# Autodesk Inventor assembly: JKSG10-95-S1
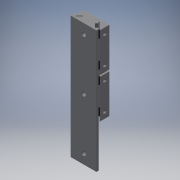
[picture p0: Inventor's stored thumbnail of the model, 180x180]
Saved by Autodesk Inventor 2019 (Build 230136000, 136)
## iProperties
Category: PARTsolutions
Company: MISUMI
Created: 2024-06-28
Part Number: JKSG10-95-S1
Catalog Web Link: www.cadenas.de
Description: JKSG, JKSC-Simplified Slide Guides for Jigs - Bearing Type Sets
Vendor: MISUMI
Document SubType Name: Assembly
Designer: psAdmin
Manufacturer: MISUMI
Mass: 13.3449 g
Surface Area: 105.666 cm^2
Volume: 13.3449 cm^3
Density: 1 g/cm^3
Title: JKSG10-95-S1
Author: Cadenas PARTsolutions
Comments: Simplified Slide Guides for Jigs - Bearing Type Sets
PSOL_IDENT_0: {$CADENAS_DATA/23d-libs/misumi/metric/07_slide_rails/jksg_asmtab.prj},205 {VTYP=3D},{STYP=ASSTAB},{N
PSOL_IDENT_1: B=JKSG10-95-S1},{LINA=JKSG10-95-S1},{NN=JKSG, JKSC},{DATE=30.06.2023 07:10:19},{GEOMDATE=09.06.2023
PSOL_IDENT_2: 02:21:08},{VERSION=},{LINEID=10},{WBVAR=TS,L,ALT,S,CALT},{WBNUMERIC=L,S,CALT}  {NB=JKSG10-95-S1},{LI
PSOL_IDENT_3: NA=JKSG10-95-S1},{KT=DUMMY},{PN=JKSG10-95-S1},{TS=SG},{L=95},{MATR=Aluminum},{MATB=Aluminum},{MATT=3
PSOL_IDENT_4: 03 Stainless Steel},{MATTP=Polyacetal},{STB=Hard Alumite Treatment},{STR=Hard Alumite Treatment},{H=
PSOL_IDENT_5: 10},{HALG=10},{A=20},{B=30},{P1=13},{P2=13},{M=3},{MALG= 'M3','M3' },{M1=3},{C=24.0},{D=6},{H1=7.5},
PSOL_IDENT_6: {E=1.8},{DGH=3.5X6X4},{N=7.5},{P=40},{MB=F682ZZ (4)},{SC=M2-5},{ALPB=49 (5)},{NOH=3},{L1=[55, 95, 13
PSOL_IDENT_7: 5, 175, 215, 255, 295, 335, 375, 415, 455, 495, 535, 575, 615]},{PPATH=jksg_asmtpl.prj},{D1=5},{D2=3
PSOL_IDENT_8: },{X=28.000},{Z=15},{W=5},{Q=8.976},{Q1=4.0},{Q2=4.976},{TIF=1},{RF=0.0},{ALT=1},{ALTALG= '','w/o Ad
PSOL_IDENT_9: ditional Sliders','1','with Additional Sliders' },{S=1},{SALG=[0:2]},{SMAX=2},{CALT=0},{CALTALG=[0:1
PSOL_IDENT_10: ]},{CALTMAX=1},{ALTPN=-S1}
NB: JKSG10-95-S1
NN: JKSG, JKSC
NT: Simplified Slide Guides for Jigs - Bearing Type Sets
NBSYN: $PN.
LINA: JKSG10-95-S1
CATALOG: Misumi
PN: JKSG10-95-S1
TS: Standard Slider Set
L: 95
MATR: Aluminum
MATB: Aluminum
MATT: 303 Stainless Steel
MATTP: Polyacetal
STB: Hard Alumite Treatment
STR: Hard Alumite Treatment
HALG: 10
A: 20
B: 30
P1: 13
P2: 13
M: 3
C: 24
D: 6
H1: 7.5
E: 1.8
DGH: 3.5X6X4
N: 7.5
P: 40
ALPB: 49 (5)
RF: 0
ALT: with Additional Sliders
S: 1
CALT: 0
SUPPLIER: MISUMI
ARTICLENO: JKSG10-95-S1
BOMINFO: JKSG10-95-S1
CREATOR: CADENAS GmbH
## Documents named in this file (4)
- e:\temp\worker_COMMON_20\temp\tmp_7460_242_rpC9F\format_0\JKSG10-95-S1.iam
- e:\temp\worker_COMMON_20\temp\tmp_7460_242_rpC9F\format_0\JKSGR10-95.ipt
- e:\temp\worker_COMMON_20\temp\tmp_7460_242_rpC9F\format_0\JKSGB10_b_b.ipt
- e:\temp\worker_COMMON_20\temp\tmp_7460_242_rpC9F\format_0\F682ZZ.ipt
## Components (11 placed, 3 different names)
1. JKSGR10-95:1
2. JKSGB10_b_b:1 — to_sc12_XY@2 <-> to_block_XY@3, to_sc12_Z@2 <-> to_block_Z@3, to_sc12_YZ@2 <-> to_block_YZ@3, tosc22_XY@2 <-> to_block_XY@4, tosc22_Z@2 <-> to_block_Z@4, tosc22_YZ@2 <-> to_block_YZ@4, to_sc1_XY@2 <-> to_block_XY@5, to_sc1_Z@2 <-> to_block_Z@5, to_sc1_YZ@2 <-> to_block_YZ@5, tosc2_XY@2 <-> to_block_XY@6, tosc2_Z@2 <-> to_block_Z@6, tosc2_YZ@2 <-> to_block_YZ@6
3. F682ZZ:1 — to_sc12_XY@2 <-> to_block_XY@3, to_sc12_Z@2 <-> to_block_Z@3, to_sc12_YZ@2 <-> to_block_YZ@3
4. F682ZZ:2 — tosc22_XY@2 <-> to_block_XY@4, tosc22_Z@2 <-> to_block_Z@4, tosc22_YZ@2 <-> to_block_YZ@4
5. F682ZZ:3 — to_sc1_XY@2 <-> to_block_XY@5, to_sc1_Z@2 <-> to_block_Z@5, to_sc1_YZ@2 <-> to_block_YZ@5
6. F682ZZ:4 — tosc2_XY@2 <-> to_block_XY@6, tosc2_Z@2 <-> to_block_Z@6, tosc2_YZ@2 <-> to_block_YZ@6
7. JKSGB10_b_b:2 — to_sc12_XY@7 <-> to_block_XY@8, to_sc12_Z@7 <-> to_block_Z@8, to_sc12_YZ@7 <-> to_block_YZ@8, tosc22_XY@7 <-> to_block_XY@9, tosc22_Z@7 <-> to_block_Z@9, tosc22_YZ@7 <-> to_block_YZ@9, to_sc1_XY@7 <-> to_block_XY@10, to_sc1_Z@7 <-> to_block_Z@10, to_sc1_YZ@7 <-> to_block_YZ@10, tosc2_XY@7 <-> to_block_XY@11, tosc2_Z@7 <-> to_block_Z@11, tosc2_YZ@7 <-> to_block_YZ@11
8. F682ZZ:5 — to_sc12_XY@7 <-> to_block_XY@8, to_sc12_Z@7 <-> to_block_Z@8, to_sc12_YZ@7 <-> to_block_YZ@8
9. F682ZZ:6 — tosc22_XY@7 <-> to_block_XY@9, tosc22_Z@7 <-> to_block_Z@9, tosc22_YZ@7 <-> to_block_YZ@9
10. F682ZZ:7 — to_sc1_XY@7 <-> to_block_XY@10, to_sc1_Z@7 <-> to_block_Z@10, to_sc1_YZ@7 <-> to_block_YZ@10
11. F682ZZ:8 — tosc2_XY@7 <-> to_block_XY@11, tosc2_Z@7 <-> to_block_Z@11, tosc2_YZ@7 <-> to_block_YZ@11
## Relationships (24: Mate 12, Angle 8, Flush 4)
- to_sc12_XY@2 <-> to_block_XY@3 [Flush]: JKSGB10_b_b:1 ↔ F682ZZ:1
- to_sc12_Z@2 <-> to_block_Z@3 [Mate]: JKSGB10_b_b:1 ↔ F682ZZ:1
- to_sc12_YZ@2 <-> to_block_YZ@3 [Angle] (0 deg): JKSGB10_b_b:1 ↔ F682ZZ:1
- tosc22_XY@2 <-> to_block_XY@4 [Flush]: JKSGB10_b_b:1 ↔ F682ZZ:2
- tosc22_Z@2 <-> to_block_Z@4 [Mate]: JKSGB10_b_b:1 ↔ F682ZZ:2
- tosc22_YZ@2 <-> to_block_YZ@4 [Angle] (0 deg): JKSGB10_b_b:1 ↔ F682ZZ:2
- to_sc1_XY@2 <-> to_block_XY@5 [Mate]: JKSGB10_b_b:1 ↔ F682ZZ:3
- to_sc1_Z@2 <-> to_block_Z@5 [Mate]: JKSGB10_b_b:1 ↔ F682ZZ:3
- to_sc1_YZ@2 <-> to_block_YZ@5 [Angle] (0 deg): JKSGB10_b_b:1 ↔ F682ZZ:3
- tosc2_XY@2 <-> to_block_XY@6 [Mate]: JKSGB10_b_b:1 ↔ F682ZZ:4
- tosc2_Z@2 <-> to_block_Z@6 [Mate]: JKSGB10_b_b:1 ↔ F682ZZ:4
- tosc2_YZ@2 <-> to_block_YZ@6 [Angle] (0 deg): JKSGB10_b_b:1 ↔ F682ZZ:4
- to_sc12_XY@7 <-> to_block_XY@8 [Flush]: JKSGB10_b_b:2 ↔ F682ZZ:5
- to_sc12_Z@7 <-> to_block_Z@8 [Mate]: JKSGB10_b_b:2 ↔ F682ZZ:5
- to_sc12_YZ@7 <-> to_block_YZ@8 [Angle] (0 deg): JKSGB10_b_b:2 ↔ F682ZZ:5
- tosc22_XY@7 <-> to_block_XY@9 [Flush]: JKSGB10_b_b:2 ↔ F682ZZ:6
- tosc22_Z@7 <-> to_block_Z@9 [Mate]: JKSGB10_b_b:2 ↔ F682ZZ:6
- tosc22_YZ@7 <-> to_block_YZ@9 [Angle] (0 deg): JKSGB10_b_b:2 ↔ F682ZZ:6
- to_sc1_XY@7 <-> to_block_XY@10 [Mate]: JKSGB10_b_b:2 ↔ F682ZZ:7
- to_sc1_Z@7 <-> to_block_Z@10 [Mate]: JKSGB10_b_b:2 ↔ F682ZZ:7
- to_sc1_YZ@7 <-> to_block_YZ@10 [Angle] (0 deg): JKSGB10_b_b:2 ↔ F682ZZ:7
- tosc2_XY@7 <-> to_block_XY@11 [Mate]: JKSGB10_b_b:2 ↔ F682ZZ:8
- tosc2_Z@7 <-> to_block_Z@11 [Mate]: JKSGB10_b_b:2 ↔ F682ZZ:8
- tosc2_YZ@7 <-> to_block_YZ@11 [Angle] (0 deg): JKSGB10_b_b:2 ↔ F682ZZ:8
